# Autodesk Inventor assembly: HS 48T Gear, No Insert
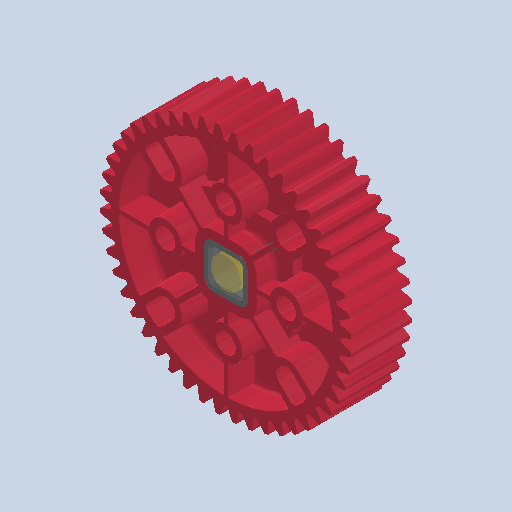
[picture p0: Inventor's stored thumbnail of the model, 512x512]
Saved by Autodesk Inventor 2025.2 (Build 292293000, 293)
## iProperties
Created: 2022-08-02
Part Number: HS 48T Gear, No Insert
Document SubType Name: Assembly
Designer: avere
Author: ylu12
## Documents named in this file (2)
- D:\vex\cad\v5\Drivetrain\Drivebay Right\HS 48T Gear, No Insert.iam
- D:\vex\cad\v5\Drivetrain\Drivebay Right\HS 48T Gear, No Insert.ipt
## Components (1 placed, 1 different names)
1. HS 48T Gear, No Insert:1 — Mate:12, Mate:11, Flush:6
## Relationships (3: Mate 2, Flush 1)
- Mate:12: HS 48T Gear, No Insert:1
- Mate:11: HS 48T Gear, No Insert:1
- Flush:6: HS 48T Gear, No Insert:1
